# Autodesk Inventor assembly: CAD Model of Bridge Assembly
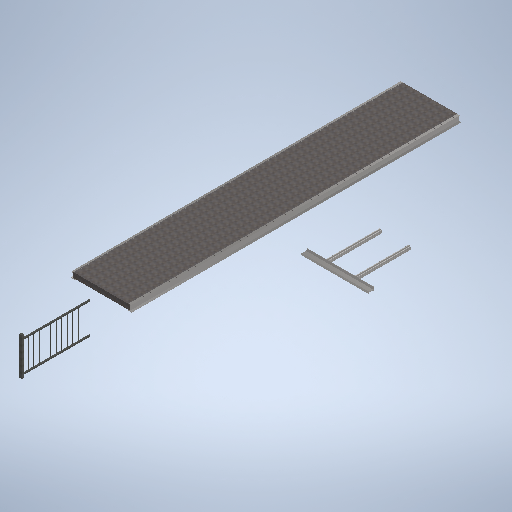
[picture p0: Inventor's stored thumbnail of the model, 512x512]
Saved by Autodesk Inventor 2025 (Build 290162000, 162)
## iProperties
Created: 2024-06-26
Part Number: CAD Model of Bridge Assembly
Document SubType Name: Assembly
Designer: track
Author: track
## Documents named in this file (6)
- C:\Users\track\OneDrive\Documents\USC-walking-bridges\Bridge_A\CAD_model\CAD Model of Bridge Assembly.iam
- C:\Users\track\OneDrive\Documents\USC-walking-bridges\Bridge_A\CAD_model\Concrete Walkway.ipt
- C:\Users\track\OneDrive\Documents\USC-walking-bridges\Bridge_A\CAD_model\Long I-Beam.ipt
- C:\Users\track\OneDrive\Documents\USC-walking-bridges\Bridge_A\CAD_model\Cylinder Supports.ipt
- C:\Users\track\OneDrive\Documents\USC-walking-bridges\Bridge_A\CAD_model\Short I-Beam.ipt
- C:\Users\track\OneDrive\Documents\USC-walking-bridges\Bridge_A\CAD_model\Railing.ipt
## Components (6 placed, 5 different names)
1. Concrete Walkway:1 — Rigid:1, Rigid:2
2. Long I-Beam:1 — Rigid:1
3. Long I-Beam:2 — Rigid:2
4. Cylinder Supports:1 — Slider:1
5. Short I-Beam:1 — Slider:1
6. Railing:1
## Relationships (3: WeldJoint 2, TranslationJoint 1)
- Rigid:1 [WeldJoint]: Concrete Walkway:1 ↔ Long I-Beam:1
- Rigid:2 [WeldJoint]: Concrete Walkway:1 ↔ Long I-Beam:2
- Slider:1 [TranslationJoint]: Cylinder Supports:1 ↔ Short I-Beam:1
